# Autodesk Inventor assembly: Assembly - v3
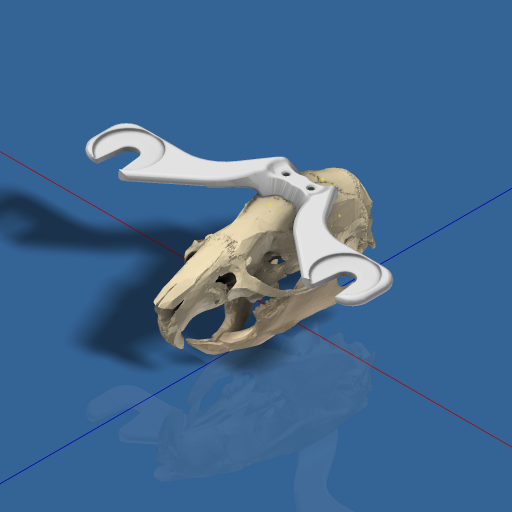
[picture p0: Inventor's stored thumbnail of the model, 512x512]
Saved by Autodesk Inventor 2024 (Build 280153000, 153)
## iProperties
Created: 2024-02-24
Part Number: Assembly - v3
Document SubType Name: Assembly
Designer: Brian
Mass: 11475.8 g
Surface Area: 143942 cm^2
Volume: 11451.8 cm^3
Density: 1.0021 g/cm^3
Author: Brian
## Documents named in this file (14)
- C:\Users\Brian\Desktop\Lab Work\Head Fixation and Probe Mounting\headplate 2024\Assembly - v4.iam
- C:\Users\Brian\Desktop\Lab Work\Head Fixation and Probe Mounting\headplate 2024\skull-95w.ipt
- C:\Users\Brian\Desktop\Lab Work\Head Fixation and Probe Mounting\headplate 2024\interface - v4.ipt
- C:\Users\Brian\Desktop\Lab Work\Head Fixation and Probe Mounting\headplate 2024\z32.ipt
- C:\Users\Brian\Desktop\Lab Work\Head Fixation and Probe Mounting\headplate 2024\zd64.ipt
- C:\Users\Brian\Desktop\Lab Work\Head Fixation and Probe Mounting\headplate 2024\screws\00-96 4-32 (1-8) 90910A440_Button Head Torx Screws.ipt
- C:\Users\Brian\Desktop\Lab Work\Head Fixation and Probe Mounting\headplate 2024\screws\00-90 4-32 (1-8) 96710A050_Stainless Steel Pan Head Torx Screws.ipt
- C:\Users\Brian\Desktop\Lab Work\Head Fixation and Probe Mounting\headplate 2024\screws\00-80 4-32 (1-8) 90910A665_Button Head Torx Screws.ipt
- C:\Users\Brian\Desktop\Lab Work\Head Fixation and Probe Mounting\headplate 2024\labrat92.ipt
- C:\Users\Brian\Desktop\Lab Work\Head Fixation and Probe Mounting\headplate 2024\0.5in_31325A27_Slip-Fit Tooling Ball with Threaded Hole.ipt
- C:\Users\Brian\Desktop\Lab Work\Head Fixation and Probe Mounting\headplate 2024\5720K27_Clamping Handle with Threaded Stud.ipt
- C:\Users\Brian\Desktop\Lab Work\Head Fixation and Probe Mounting\headplate 2024\B3048F-thorlabs-airtable-breadboard.ipt
- C:\Users\Brian\Desktop\Lab Work\Head Fixation and Probe Mounting\headplate 2024\91197A480_316 Stainless Steel Male-Female Threaded Hex Standoff.ipt
- C:\Users\Brian\Desktop\Lab Work\Head Fixation and Probe Mounting\headplate 2024\5720K25_Clamping Handle with Threaded Stud.ipt
## Components (19 placed, 18 different names)
1. skull-95w:1 — Flush:1, Flush:2, Flush:3, Mate:1, Mate:3, Mate:4, Mate:5, Angle:1, Mate:8, Mate:9, Mate:10, Mate:11, Mate:12, Mate:13
2. zd64:PFC-L — Mate:8
3. zd64:PFC-R — Mate:4
4. zd64:IC-L — Mate:9
5. zd64:IC-R — Mate:10
6. zd64:AC-L — Mate:5, Angle:1
7. zd64:AC-R — Mate:11
8. z32:1 — Mate:3
9. interface - v4:1 — Flush:1, Flush:2, Flush:3, Mate:1, Mate:14, Insert:3, Insert:4
10. 00-96 4-32 (1-8) 90910A440_Button Head Torx Screws:1 — Mate:14
11. 00-90 4-32 (1-8) 96710A050_Stainless Steel Pan Head Torx Screws:1 — Insert:4
12. 00-80 4-32 (1-8) 90910A665_Button Head Torx Screws:1 — Insert:3
13. labrat92:1
14. 0.5in_31325A27_Slip-Fit Tooling Ball with Threaded Hole:1
15. 5720K27_Clamping Handle with Threaded Stud:2
16. B3048F-thorlabs-airtable-breadboard:1 — Insert:2
17. 91197A480_316 Stainless Steel Male-Female Threaded Hex Standoff:1 — Insert:1
18. 5720K25_Clamping Handle with Threaded Stud:1
19. 91197A480_316 Stainless Steel Male-Female Threaded Hex Standoff:2 — Insert:1, Insert:2
## Relationships (20: Mate 11, Insert 4, Flush 3, Angle 2)
- Flush:1: skull-95w:1 ↔ interface - v4:1
- Flush:2: skull-95w:1 ↔ interface - v4:1
- Flush:3: skull-95w:1 ↔ interface - v4:1
- Mate:1: skull-95w:1 ↔ interface - v4:1
- Mate:3: skull-95w:1 ↔ z32:1
- Mate:4: skull-95w:1 ↔ zd64:PFC-R
- Mate:5: skull-95w:1 ↔ zd64:AC-L
- Angle:1 (180 deg): skull-95w:1 ↔ zd64:AC-L
- Mate:8: skull-95w:1 ↔ zd64:PFC-L
- Mate:9: skull-95w:1 ↔ zd64:IC-L
- Mate:10: skull-95w:1 ↔ zd64:IC-R
- Mate:11: skull-95w:1 ↔ zd64:AC-R
- Mate:12: skull-95w:1
- Mate:13: skull-95w:1
- Angle:3 (0 deg)
- Mate:14: interface - v4:1 ↔ 00-96 4-32 (1-8) 90910A440_Button Head Torx Screws:1
- Insert:1: 91197A480_316 Stainless Steel Male-Female Threaded Hex Standoff:1 ↔ 91197A480_316 Stainless Steel Male-Female Threaded Hex Standoff:2
- Insert:2 (-10 mm): B3048F-thorlabs-airtable-breadboard:1 ↔ 91197A480_316 Stainless Steel Male-Female Threaded Hex Standoff:2
- Insert:3: interface - v4:1 ↔ 00-80 4-32 (1-8) 90910A665_Button Head Torx Screws:1
- Insert:4: interface - v4:1 ↔ 00-90 4-32 (1-8) 96710A050_Stainless Steel Pan Head Torx Screws:1
